# Autodesk Inventor assembly: Mohne komplett
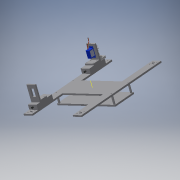
[picture p0: Inventor's stored thumbnail of the model, 180x180]
Saved by Autodesk Inventor 2018 (Build 220112000, 112)
## iProperties
Created: 2018-01-26
Part Number: Mohne komplett
Material: Generisch
Document SubType Name: Assembly
Designer: fhinstall
Author: fhinstall
## Documents named in this file (13)
- C:\Users\gchri\OneDrive\Development\RTW\03_Konstruktion\Mohne komplett.iam
- C:\Users\gchri\OneDrive\Development\RTW\03_Konstruktion\Metall Stab M5.ipt
- C:\Users\gchri\OneDrive\Development\RTW\03_Konstruktion\zweites Teil rotorachse.ipt
- C:\Users\gchri\OneDrive\Development\RTW\03_Konstruktion\Gegenstück Rotorachse.ipt
- C:\Users\gchri\OneDrive\Development\RTW\03_Konstruktion\L-Halterung Servo.ipt
- C:\Users\gchri\OneDrive\Development\RTW\03_Konstruktion\chassis mit motorlöcher.ipt
- C:\Users\gchri\OneDrive\Development\RTW\03_Konstruktion\Platzhalter Zylinder Klein.ipt
- C:\Users\gchri\OneDrive\Development\RTW\03_Konstruktion\L-Halterung Servo_MIR.ipt
- C:\Users\gchri\OneDrive\Development\RTW\03_Konstruktion\Gegenstück Rotorachse_MIR.ipt
- C:\Users\gchri\OneDrive\Development\RTW\03_Konstruktion\zweites Teil rotorachse_MIR.ipt
- C:\Users\gchri\OneDrive\Development\RTW\03_Konstruktion\Metall Stab M5_MIR.ipt
- C:\Users\gchri\OneDrive\Development\RTW\03_Konstruktion\Chassis-2.ipt
- C:\Users\gchri\OneDrive\Development\RTW\03_Konstruktion\StirnradUNDServo.iam
## Components (15 placed, 12 different names)
1. chassis mit motorlöcher:1 — Passend:4, Fluchtend:7, Fluchtend:8, Passend:6, Fluchtend:11, Fluchtend:12, Drehbar:1, Drehbar:2, Starr:1, Drehbar:3, Passend:7, Winkel:1, Passend:9, Fluchtend:15, Fluchtend:16, Passend:10, Fluchtend:17, Fluchtend:18
2. L-Halterung Servo:2 — Passend:5, Fluchtend:9, Fluchtend:10
3. Gegenstück Rotorachse:2 — Passend:4, Fluchtend:7, Fluchtend:8, Passend:5, Fluchtend:9, Fluchtend:10, Zylindrisch:2
4. zweites Teil rotorachse:2 — Passend:6, Fluchtend:11, Fluchtend:12
5. Metall Stab M5:2 — Zylindrisch:2
6. Platzhalter Zylinder Klein:1 — Drehbar:2
7. Platzhalter Zylinder Klein:2 — Starr:1, Drehbar:4
8. Platzhalter Zylinder Klein:3 — Drehbar:1
9. Platzhalter Zylinder Klein:4 — Drehbar:3, Drehbar:5
10. L-Halterung Servo_MIR:1 — Fluchtend:13, Fluchtend:14, Passend:8, Passend:12, Passend:13
11. Gegenstück Rotorachse_MIR:1 — Fluchtend:13, Fluchtend:14, Passend:8, Zylindrisch:3, Passend:9, Fluchtend:15, Fluchtend:16
12. zweites Teil rotorachse_MIR:1 — Passend:10, Fluchtend:17, Fluchtend:18
13. Metall Stab M5_MIR:1 — Zylindrisch:3
14. Chassis-2:1 — Drehbar:4, Drehbar:5
15. StirnradUNDServo:1 [sub-assembly] — Passend:12, Passend:13
## Relationships (30: Flush 12, Mate 9, RevoluteJoint 5, CylindricalJoint 2, WeldJoint 1, Angle 1)
- Passend:4 [Mate]: chassis mit motorlöcher:1 ↔ Gegenstück Rotorachse:2
- Fluchtend:7 [Flush] (40 mm): chassis mit motorlöcher:1 ↔ Gegenstück Rotorachse:2
- Fluchtend:8 [Flush]: chassis mit motorlöcher:1 ↔ Gegenstück Rotorachse:2
- Passend:5 [Mate]: L-Halterung Servo:2 ↔ Gegenstück Rotorachse:2
- Fluchtend:9 [Flush]: L-Halterung Servo:2 ↔ Gegenstück Rotorachse:2
- Fluchtend:10 [Flush]: L-Halterung Servo:2 ↔ Gegenstück Rotorachse:2
- Passend:6 [Mate]: chassis mit motorlöcher:1 ↔ zweites Teil rotorachse:2
- Fluchtend:11 [Flush]: chassis mit motorlöcher:1 ↔ zweites Teil rotorachse:2
- Fluchtend:12 [Flush] (25 mm): chassis mit motorlöcher:1 ↔ zweites Teil rotorachse:2
- Zylindrisch:2 [CylindricalJoint]: Gegenstück Rotorachse:2 ↔ Metall Stab M5:2
- Drehbar:1 [RevoluteJoint]: chassis mit motorlöcher:1 ↔ Platzhalter Zylinder Klein:3
- Drehbar:2 [RevoluteJoint]: chassis mit motorlöcher:1 ↔ Platzhalter Zylinder Klein:1
- Starr:1 [WeldJoint]: chassis mit motorlöcher:1 ↔ Platzhalter Zylinder Klein:2
- Drehbar:3 [RevoluteJoint]: chassis mit motorlöcher:1 ↔ Platzhalter Zylinder Klein:4
- Passend:7 [Mate]: chassis mit motorlöcher:1
- Winkel:1 [Angle] (90 deg): chassis mit motorlöcher:1
- Fluchtend:13 [Flush]: L-Halterung Servo_MIR:1 ↔ Gegenstück Rotorachse_MIR:1
- Fluchtend:14 [Flush]: L-Halterung Servo_MIR:1 ↔ Gegenstück Rotorachse_MIR:1
- Passend:8 [Mate]: L-Halterung Servo_MIR:1 ↔ Gegenstück Rotorachse_MIR:1
- Zylindrisch:3 [CylindricalJoint]: Gegenstück Rotorachse_MIR:1 ↔ Metall Stab M5_MIR:1
- Passend:9 [Mate]: chassis mit motorlöcher:1 ↔ Gegenstück Rotorachse_MIR:1
- Fluchtend:15 [Flush]: chassis mit motorlöcher:1 ↔ Gegenstück Rotorachse_MIR:1
- Fluchtend:16 [Flush] (-40 mm): chassis mit motorlöcher:1 ↔ Gegenstück Rotorachse_MIR:1
- Passend:10 [Mate]: chassis mit motorlöcher:1 ↔ zweites Teil rotorachse_MIR:1
- Fluchtend:17 [Flush]: chassis mit motorlöcher:1 ↔ zweites Teil rotorachse_MIR:1
- Fluchtend:18 [Flush] (25 mm): chassis mit motorlöcher:1 ↔ zweites Teil rotorachse_MIR:1
- Drehbar:4 [RevoluteJoint]: Platzhalter Zylinder Klein:2 ↔ Chassis-2:1
- Drehbar:5 [RevoluteJoint]: Platzhalter Zylinder Klein:4 ↔ Chassis-2:1
- Passend:12 [Mate]: L-Halterung Servo_MIR:1 ↔ StirnradUNDServo:1
- Passend:13 [Mate]: L-Halterung Servo_MIR:1 ↔ StirnradUNDServo:1
